# Autodesk Inventor assembly: manual shifter and A bot gearbox
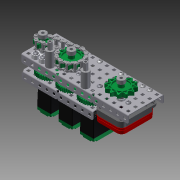
[picture p0: Inventor's stored thumbnail of the model, 180x180]
Saved by Autodesk Inventor 2014 SP1 (Build 180222100, 222)
## iProperties
Created: 2013-08-29
Part Number: manual shifter and A bot gearbox
Document SubType Name: Assembly
Designer: Ryan
Sending System: SolidWorks 2013
Last Author: Ryan
Author: Ryan
## Documents named in this file (3)
- C:\Users\Ryan\Desktop\sw\toss up 1st A bot\inventor drive\manual shifter and A bot gearbox.iam
- C:\Users\Ryan\Desktop\sw\toss up 1st A bot\inventor drive\manual shifter.iam
- C:\Users\Ryan\Desktop\sw\toss up 1st A bot\inventor drive\toss up A bot gearbox.iam
## Components (2 placed, 2 different names)
1. toss up A bot gearbox:1 [sub-assembly] — Flush:1, Flush:2, Mate:1
2. manual shifter:1 [sub-assembly] — Flush:1, Flush:2, Mate:1
## Relationships (3: Flush 2, Mate 1)
- Flush:1: toss up A bot gearbox:1 ↔ manual shifter:1
- Flush:2: toss up A bot gearbox:1 ↔ manual shifter:1
- Mate:1 (25.4 mm): toss up A bot gearbox:1 ↔ manual shifter:1
